# Autodesk Inventor assembly: MectoSYS
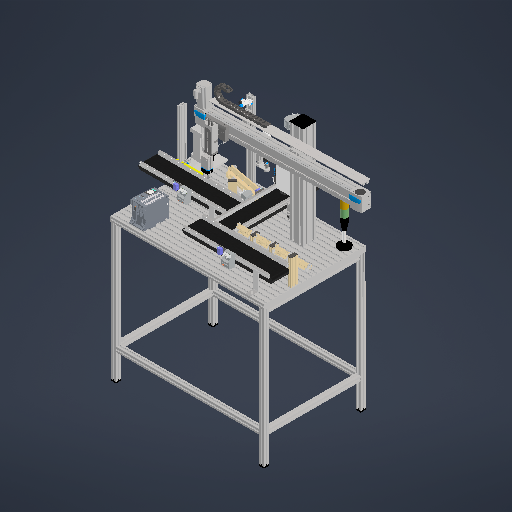
[picture p0: Inventor's stored thumbnail of the model, 512x512]
Saved by Autodesk Inventor 2027 (Build 310192000, 192)
## iProperties
Created: 2026-04-15
Part Number: MectoSYS
Document SubType Name: Assembly
Designer: ratik
Author: ratik
## Documents named in this file (9)
- C:\Users\ratik\OneDrive\Personal Folder\00_Startup\01_Mectosys_Prototype\01_Prototype\01_Mechanical\3D file\Assembly File\MectoSYS.iam
- C:\Users\ratik\OneDrive\Personal Folder\00_Startup\01_Mectosys_Prototype\01_Prototype\01_Mechanical\3D file\Assembly File\Base assembly.iam
- C:\Users\ratik\OneDrive\Personal Folder\00_Startup\01_Mectosys_Prototype\01_Prototype\01_Mechanical\3D file\Assembly File\Slider.iam
- C:\Users\ratik\OneDrive\Personal Folder\00_Startup\01_Mectosys_Prototype\01_Prototype\01_Mechanical\3D file\Assembly File\Conveyor Module.iam
- C:\Users\ratik\OneDrive\Personal Folder\00_Startup\01_Mectosys_Prototype\01_Prototype\01_Mechanical\3D file\Assembly File\Handlling Module.iam
- C:\Users\ratik\OneDrive\Personal Folder\00_Startup\01_Mectosys_Prototype\01_Prototype\01_Mechanical\3D file\Assembly File\Pick and place module.iam
- C:\Users\ratik\OneDrive\Personal Folder\00_Startup\01_Mectosys_Prototype\01_Prototype\01_Mechanical\3D file\Assembly File\Distribution module.iam
- C:\Users\ratik\OneDrive\Personal Folder\00_Startup\01_Mectosys_Prototype\01_Prototype\01_Mechanical\3D file\07_Comp\led-stack-light-indicator-signal-1.snapshot.3\Stack Light\Assembly Light Stack.iam
- C:\Users\ratik\Downloads\plc-s7-1500-model-6es7511-1ck00-0ab0-1.snapshot.1\6es75111ck000ab0\6es75111ck000ab0.ipt
## Components (13 placed, 8 different names)
1. Base assembly:1 [sub-assembly] — Mate:3, Mate:4, Mate:6, Mate:7, Mate:8, Mate:9, Mate:11, Mate:12, Mate:13, Mate:14, Mate:15, Mate:16
2. Conveyor Module:1 [sub-assembly] — Mate:6
3. Conveyor Module:2 [sub-assembly] — Mate:8
4. Conveyor Module:3 [sub-assembly] — Mate:7
5. Handlling Module:1 [sub-assembly] — Mate:9, Mate:11
6. Pick and place module:1 [sub-assembly] — Mate:12
7. Slider:4 [sub-assembly] — Mate:13
8. Distribution module:1 [sub-assembly] — Mate:14
9. Assembly Light Stack:1 [sub-assembly] — Mate:15
10. 6es75111ck000ab0:1 — Mate:16
11. Slider:1 [sub-assembly] — Mate:3
12. Slider:2 [sub-assembly]
13. Slider:3 [sub-assembly] — Mate:4
## Component patterns: (3 elements, first: Slider:1)
## Relationships (12: Mate 12)
- Mate:3: Base assembly:1 ↔ Slider:1
- Mate:4 (-680 mm): Base assembly:1 ↔ Slider:3
- Mate:6: Base assembly:1 ↔ Conveyor Module:1
- Mate:7: Base assembly:1 ↔ Conveyor Module:3
- Mate:8: Base assembly:1 ↔ Conveyor Module:2
- Mate:9: Base assembly:1 ↔ Handlling Module:1
- Mate:11: Base assembly:1 ↔ Handlling Module:1
- Mate:12: Base assembly:1 ↔ Pick and place module:1
- Mate:13: Base assembly:1 ↔ Slider:4
- Mate:14: Base assembly:1 ↔ Distribution module:1
- Mate:15: Base assembly:1 ↔ Assembly Light Stack:1
- Mate:16: Base assembly:1 ↔ 6es75111ck000ab0:1
